# Autodesk Inventor assembly: Plate 1
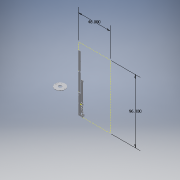
[picture p0: Inventor's stored thumbnail of the model, 180x180]
Saved by Autodesk Inventor 2016 (Build 200138000, 138)
## iProperties
Created: 2016-04-26
Part Number: Plate 1
Document SubType Name: Assembly
Designer: rubenjm
Author: rubenjm
## Documents named in this file (10)
- C:\Users\rubenjm\Documents\To Transfer\2k16 Spring\RME\GGC\V3\Plate 1.iam
- C:\Users\rubenjm\Documents\To Transfer\2k16 Spring\RME\GGC\V3\Arm Base.ipt
- C:\Users\rubenjm\Documents\To Transfer\2k16 Spring\RME\GGC\V3\Holder.ipt
- C:\Users\rubenjm\Documents\To Transfer\2k16 Spring\RME\GGC\V3\Far End Cap.ipt
- C:\Users\rubenjm\Documents\To Transfer\2k16 Spring\RME\GGC\V3\Near Holder.ipt
- C:\Users\rubenjm\Documents\To Transfer\2k16 Spring\RME\GGC\V3\Motor Bracket.ipt
- C:\Users\rubenjm\Documents\To Transfer\2k16 Spring\RME\GGC\V3\Near End Cap.ipt
- C:\Users\rubenjm\Documents\To Transfer\2k16 Spring\RME\GGC\V3\Arm Side.ipt
- C:\Users\rubenjm\Documents\To Transfer\2k16 Spring\RME\GGC\V3\Arm Top.ipt
- C:\Users\rubenjm\Documents\To Transfer\2k16 Spring\RME\GGC\V3\Turntable Top.ipt
## Components (11 placed, 9 different names)
1. Arm Base:1 — Mate:1, Mate:2, Mate:3, Mate:6, Mate:12, Mate:19, Mate:22, Mate:24, Mate:26, Mate:32
2. Holder:1 — Mate:4, Mate:6, Mate:8, Mate:9, Mate:14
3. Holder:2 — Mate:7, Mate:8, Mate:9, Mate:11
4. Far End Cap:1 — Mate:10, Mate:11, Mate:12, Mate:15, Mate:16
5. Near Holder:1 — Mate:13, Mate:15, Mate:16, Mate:18
6. Motor Bracket:1 — Mate:17, Mate:18, Mate:19, Mate:20
7. Near End Cap:1 — Mate:20, Mate:21, Mate:22, Mate:31
8. Arm Side:1 — Mate:24, Mate:25, Mate:26, Mate:27, Mate:29
9. Arm Side:2 — Mate:27, Mate:28, Mate:29
10. Arm Top:1 — Mate:30, Mate:31, Mate:32
11. Turntable Top:1
## Relationships (30: Mate 30)
- Mate:1: Arm Base:1
- Mate:2 (6.35 mm): Arm Base:1
- Mate:3 (6.35 mm): Arm Base:1
- Mate:4: Holder:1
- Mate:6 (6.35 mm): Arm Base:1 ↔ Holder:1
- Mate:7: Holder:2
- Mate:8 (6.35 mm): Holder:1 ↔ Holder:2
- Mate:9 (6.35 mm): Holder:1 ↔ Holder:2
- Mate:10: Far End Cap:1
- Mate:11 (6.35 mm): Holder:2 ↔ Far End Cap:1
- Mate:12 (6.35 mm): Arm Base:1 ↔ Far End Cap:1
- Mate:13: Near Holder:1
- Mate:14: Holder:1
- Mate:15 (6.35 mm): Far End Cap:1 ↔ Near Holder:1
- Mate:16 (6.35 mm): Far End Cap:1 ↔ Near Holder:1
- Mate:17: Motor Bracket:1
- Mate:18 (6.35 mm): Near Holder:1 ↔ Motor Bracket:1
- Mate:19 (6.35 mm): Arm Base:1 ↔ Motor Bracket:1
- Mate:20 (6.35 mm): Motor Bracket:1 ↔ Near End Cap:1
- Mate:21: Near End Cap:1
- Mate:22 (6.35 mm): Arm Base:1 ↔ Near End Cap:1
- Mate:24 (6.35 mm): Arm Base:1 ↔ Arm Side:1
- Mate:25: Arm Side:1
- Mate:26: Arm Base:1 ↔ Arm Side:1
- Mate:27: Arm Side:1 ↔ Arm Side:2
- Mate:28: Arm Side:2
- Mate:29 (6.35 mm): Arm Side:1 ↔ Arm Side:2
- Mate:30: Arm Top:1
- Mate:31 (6.35 mm): Near End Cap:1 ↔ Arm Top:1
- Mate:32 (6.35 mm): Arm Base:1 ↔ Arm Top:1
